# Autodesk Inventor assembly: Baugruppe_Montage_Ring_Vorne
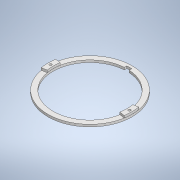
[picture p0: Inventor's stored thumbnail of the model, 180x180]
Saved by Autodesk Inventor 2022.2 (Build 262287010, 287A)
## iProperties
Created: 2024-01-10
Part Number: Baugruppe_Montage_Ring_Vorne
Document SubType Name: Assembly
Designer: ppovolni
Author: ppovolni
## Documents named in this file (4)
- D:\3_Local_Projekte\_PaperGitHub\MiniBumblebee_LowFieldMapping\2_Calibration\21_Hardware\213_CalibrationSolenoid_CAD\Cylinder\ASM_Mounting_Ring_Front.iam
- D:\3_Local_Projekte\_PaperGitHub\MiniBumblebee_LowFieldMapping\2_Calibration\21_Hardware\213_CalibrationSolenoid_CAD\Cylinder\Mounting_Ring_Front.ipt
- D:\3_Local_Projekte\_PaperGitHub\MiniBumblebee_LowFieldMapping\2_Calibration\21_Hardware\213_CalibrationSolenoid_CAD\Cylinder\Mounting_Ring_Front_Thickening.ipt
- D:\3_Local_Projekte\_PaperGitHub\MiniBumblebee_LowFieldMapping\2_Calibration\21_Hardware\213_CalibrationSolenoid_CAD\Cylinder\Mounting_Ring_Front_Thickening_MIR.ipt
## Components (3 placed, 3 different names)
1. Mounting_Ring_Front:1 — Fluchtend:1, Fluchtend:2
2. Mounting_Ring_Front_Thickening:1 — Fluchtend:1, Fluchtend:2
3. Mounting_Ring_Front_Thickening_MIR:1
## Relationships (2: Flush 2)
- Fluchtend:1 [Flush]: Mounting_Ring_Front:1 ↔ Mounting_Ring_Front_Thickening:1
- Fluchtend:2 [Flush]: Mounting_Ring_Front:1 ↔ Mounting_Ring_Front_Thickening:1
